# Autodesk Inventor assembly: Baugruppe1
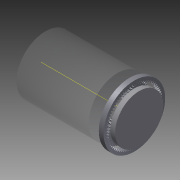
[picture p0: Inventor's stored thumbnail of the model, 180x180]
Saved by Autodesk Inventor 2014 (Build 180170000, 170)
## iProperties
Created: 2013-05-23
Part Number: Baugruppe1
Document SubType Name: Assembly
Designer: hartmann
Author: hartmann
## Documents named in this file (6)
- C:\Dokumente und Einstellungen\hartmann\Desktop\Beep\Hardware\Model\Baugruppe1.iam
- C:\Dokumente und Einstellungen\hartmann\Desktop\Beep\Hardware\Model\motor.ipt
- C:\Dokumente und Einstellungen\hartmann\Desktop\Beep\Hardware\Model\Baugruppe1\Konstruktions-Assistent\Stirnräder1.iam
- C:\Dokumente und Einstellungen\hartmann\Desktop\Beep\Hardware\Model\Baugruppe1\Konstruktions-Assistent\Stirnräder2.iam
- C:\Dokumente und Einstellungen\hartmann\Desktop\Beep\Hardware\Model\Baugruppe1\Konstruktions-Assistent\Stirnräder3.iam
- C:\Dokumente und Einstellungen\hartmann\Desktop\Beep\Hardware\Model\PSteg.ipt
## Components (7 placed, 3 different names)
1. motor:1 — Passend:1, Passend:2
2. Stirnräder:1 [sub-assembly] — Passend:2, Passend:3, Fluchtend:2, Fluchtend:3, Fluchtend:4
3. Stirnräder:3 [sub-assembly] — Fluchtend:2, Passend:4
4. PSteg:1 — Fluchtend:4
5. Stirnräder:2 [sub-assembly] — Passend:5, Fluchtend:3
6. Stirnräder:4 [sub-assembly]
7. Stirnräder:5 [sub-assembly]
## Component patterns: (3 elements, first: Stirnräder:2)
## Relationships (8: Mate 5, Flush 3)
- Passend:1 [Mate]: motor:1
- Passend:2 [Mate] (5 mm): motor:1 ↔ Stirnräder:1
- Passend:3 [Mate]: Stirnräder:1
- Fluchtend:2 [Flush]: Stirnräder:1 ↔ Stirnräder:3
- Passend:4 [Mate]: Stirnräder:3
- Passend:5 [Mate] (6.75 mm): Stirnräder:2
- Fluchtend:3 [Flush]: Stirnräder:1 ↔ Stirnräder:2
- Fluchtend:4 [Flush]: Stirnräder:1 ↔ PSteg:1
